# Autodesk Inventor assembly: Raspberry Pi 4 Complete
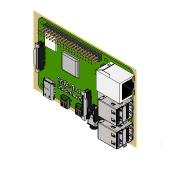
[picture p0: Inventor's stored thumbnail of the model, 180x180]
Saved by Autodesk Inventor 2020 (Build 240168000, 168)
## iProperties
Created: 2020-02-12
Part Number: Raspberry Pi 4 Complete
Document SubType Name: Assembly
Designer: ahamm
Author: ahamm
## Documents named in this file (5)
- C:\Users\ahamm\Desktop\Inventor 2020 Parts\Inventor Download\Raspberry Pi 4 Complete.iam
- C:\Users\ahamm\Desktop\Inventor 2020 Parts\Inventor Download\raspberry_p4b_v001.ipt
- C:\Users\ahamm\Desktop\Inventor 2020 Parts\Inventor Download\SoC.ipt
- C:\Users\ahamm\Desktop\Inventor 2020 Parts\Inventor Download\WiFi.ipt
- C:\Users\ahamm\Desktop\Inventor 2020 Parts\Inventor Download\indiceuk.ipt
## Components (4 placed, 4 different names)
1. raspberry_p4b_v001:1 — Flush:1, Flush:2, Flush:3, Flush:4, Flush:5, Flush:6
2. SoC:1 — Flush:1, Flush:2
3. WiFi:1 — Flush:3, Flush:4
4. indiceuk:1 — Flush:5, Flush:6
## Relationships (6: Flush 6)
- Flush:1: raspberry_p4b_v001:1 ↔ SoC:1
- Flush:2: raspberry_p4b_v001:1 ↔ SoC:1
- Flush:3: raspberry_p4b_v001:1 ↔ WiFi:1
- Flush:4: raspberry_p4b_v001:1 ↔ WiFi:1
- Flush:5: raspberry_p4b_v001:1 ↔ indiceuk:1
- Flush:6: raspberry_p4b_v001:1 ↔ indiceuk:1
